# Autodesk Inventor assembly: MotorPhotogateAssembly
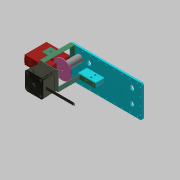
[picture p0: Inventor's stored thumbnail of the model, 180x180]
Saved by Autodesk Inventor 2018 (Build 220112000, 112)
## iProperties
Created: 2019-07-16
Part Number: MotorPhotogateAssembly
Document SubType Name: Assembly
Designer: mkivekas
Author: mkivekas
## Documents named in this file (7)
- \\cern.ch\dfs\Users\m\mkivekas\Documents\Inventor\MotorPhotogateAssembly.iam
- \\cern.ch\dfs\Users\m\mkivekas\Documents\Inventor\MotorSupport.ipt
- \\cern.ch\dfs\Users\m\mkivekas\Documents\Inventor\PhotogateCover.ipt
- \\cern.ch\dfs\Users\m\mkivekas\Documents\Inventor\RotatoryDisk.ipt
- \\cern.ch\dfs\Users\m\mkivekas\Documents\Inventor\PAC-SLI\Furnace drive block\PAC-SLI furnace Rv6 base.ipt
- \\cern.ch\dfs\Users\m\mkivekas\Documents\Inventor\Cylinder.ipt
- \\cern.ch\dfs\Users\m\mkivekas\Documents\Inventor\QSH4218-35rev2.ipt
## Components (6 placed, 6 different names)
1. MotorSupport:1 — Mate:2, Mate:3, Mate:4, Mate:5
2. PhotogateCover:1
3. RotatoryDisk:1
4. PAC-SLI furnace Rv6 base:1 — Mate:2
5. Cylinder:1
6. QSH4218-35rev2:1 — Mate:3, Mate:4, Mate:5
## Relationships (4: Mate 4)
- Mate:2: MotorSupport:1 ↔ PAC-SLI furnace Rv6 base:1
- Mate:3: MotorSupport:1 ↔ QSH4218-35rev2:1
- Mate:4: MotorSupport:1 ↔ QSH4218-35rev2:1
- Mate:5: MotorSupport:1 ↔ QSH4218-35rev2:1
